# Autodesk Inventor assembly: J008644
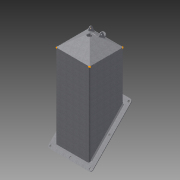
[picture p0: Inventor's stored thumbnail of the model, 180x180]
Saved by Autodesk Inventor 2020.3 (Build 243373000, 373)
## iProperties
Created: 2020-09-10
Part Number: J008644
Vendor: HHMI: JRC - ID&F
Document SubType Name: Weldment
Designer: talbotj
Weld Material: STAINLESS STEEL, 316
Description: FULL WELDMENT FOR RAT CAGE BOTTLE HOLDER V4
Project: P-342901
ALTERED ITEM DESCRIPTION: N/A
ALTERED ITEM PART NUMBER: N/A
ALTERED ITEM VENDOR: N/A
DESIGN DEPARTMENT: HHMI: JRC - ID&F
LAB/DEPT: VIVARIUM (SHARED RESOURCES)
REQUESTING SCIENTIST: COX, JAMES
SPECIAL FINISH: N/A
SURFACE ROUGHNESS: N/A
Author: talbotj
Revision Number: A
## Documents named in this file (6)
- C:\_WORKSPACE\DATA\PROJECTS\_PROJECTS BY LAB\VIVARIUM\RAT CAGE MODIFICATIONS\RCBH4\RCBH4 WELDMENT.iam
- C:\_WORKSPACE\DATA\PROJECTS\_PROJECTS BY LAB\VIVARIUM\RAT CAGE MODIFICATIONS\RCBH4\RCBH4 CONE.ipt
- C:\_WORKSPACE\DATA\PROJECTS\_PROJECTS BY LAB\VIVARIUM\RAT CAGE MODIFICATIONS\RCBH4\RCBH4 FLAP HOLDER.ipt
- C:\_WORKSPACE\DATA\PROJECTS\_PROJECTS BY LAB\VIVARIUM\RAT CAGE MODIFICATIONS\RCBH4\RCBH4 WALLS A.ipt
- C:\_WORKSPACE\DATA\PROJECTS\_PROJECTS BY LAB\VIVARIUM\RAT CAGE MODIFICATIONS\RCBH4\RCBH4 WALLS B.ipt
- C:\_WORKSPACE\DATA\PROJECTS\_PROJECTS BY LAB\VIVARIUM\RAT CAGE MODIFICATIONS\RCBH4\RCBH4 MOUNT PLATE.ipt
## Components (6 placed, 5 different names)
1. RCBH4 CONE:1 — Flush:3, Mate:5, Mate:6, Flush:4, Mate:7, Mate:9, Flush:5
2. RCBH4 FLAP HOLDER:1 — Mate:9, Flush:5
3. RCBH4 WALLS A:1 — Flush:1, Mate:1, Mate:2, Flush:4, Mate:10
4. RCBH4 WALLS B:1 — Flush:1, Mate:1, Mate:2, Mate:3, Flush:2, Mate:7, Mate:8
5. RCBH4 CONE:2 — Flush:3, Mate:5, Mate:6, Mate:8
6. RCBH4 MOUNT PLATE:1 — Mate:3, Flush:2, Mate:10
## Relationships (14: Mate 9, Flush 5)
- Flush:1: RCBH4 WALLS A:1 ↔ RCBH4 WALLS B:1
- Mate:1: RCBH4 WALLS A:1 ↔ RCBH4 WALLS B:1
- Mate:2: RCBH4 WALLS A:1 ↔ RCBH4 WALLS B:1
- Mate:3: RCBH4 WALLS B:1 ↔ RCBH4 MOUNT PLATE:1
- Flush:2: RCBH4 WALLS B:1 ↔ RCBH4 MOUNT PLATE:1
- Flush:3: RCBH4 CONE:1 ↔ RCBH4 CONE:2
- Mate:5: RCBH4 CONE:1 ↔ RCBH4 CONE:2
- Mate:6: RCBH4 CONE:1 ↔ RCBH4 CONE:2
- Flush:4: RCBH4 CONE:1 ↔ RCBH4 WALLS A:1
- Mate:7: RCBH4 CONE:1 ↔ RCBH4 WALLS B:1
- Mate:8: RCBH4 WALLS B:1 ↔ RCBH4 CONE:2
- Mate:9: RCBH4 CONE:1 ↔ RCBH4 FLAP HOLDER:1
- Flush:5 (8.636 mm): RCBH4 CONE:1 ↔ RCBH4 FLAP HOLDER:1
- Mate:10: RCBH4 WALLS A:1 ↔ RCBH4 MOUNT PLATE:1
